# Autodesk Inventor assembly: New Exhaust Assembled
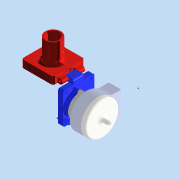
[picture p0: Inventor's stored thumbnail of the model, 180x180]
Saved by Autodesk Inventor 2020 (Build 240168000, 168)
## iProperties
Created: 2020-04-10
Part Number: New Exhaust Assembled
Document SubType Name: Assembly
Designer: Simon
Author: Simon
## Documents named in this file (5)
- D:\GrabCAD\MTL Ventilator Design\Filter housing with o ring\New Exhaust Assembled.iam
- D:\GrabCAD\MTL Ventilator Design\Filter housing with o ring\NewExhaustValve.iam
- D:\GrabCAD\MTL Ventilator Design\Filter housing with o ring\clip.ipt
- D:\GrabCAD\MTL Ventilator Design\Filter housing with o ring\filter_connector v1 (1).ipt
- D:\GrabCAD\MTL Ventilator Design\Filter housing with o ring\exhaustCap.ipt
## Components (4 placed, 4 different names)
1. NewExhaustValve:1 [sub-assembly] — Mate:1, Mate:2, Mate:3, Mate:4, Mate:5, Mate:6, Mate:7
2. clip:1 — Mate:3, Mate:4, Mate:5
3. filter_connector v1 (1):1 — Mate:1, Mate:2
4. exhaustCap:1 — Mate:6, Mate:7
## Relationships (7: Mate 7)
- Mate:1: NewExhaustValve:1 ↔ filter_connector v1 (1):1
- Mate:2 (0.2 mm): NewExhaustValve:1 ↔ filter_connector v1 (1):1
- Mate:3: NewExhaustValve:1 ↔ clip:1
- Mate:4: NewExhaustValve:1 ↔ clip:1
- Mate:5: NewExhaustValve:1 ↔ clip:1
- Mate:6: NewExhaustValve:1 ↔ exhaustCap:1
- Mate:7: NewExhaustValve:1 ↔ exhaustCap:1
